# Autodesk Inventor assembly: load_cell_assembly
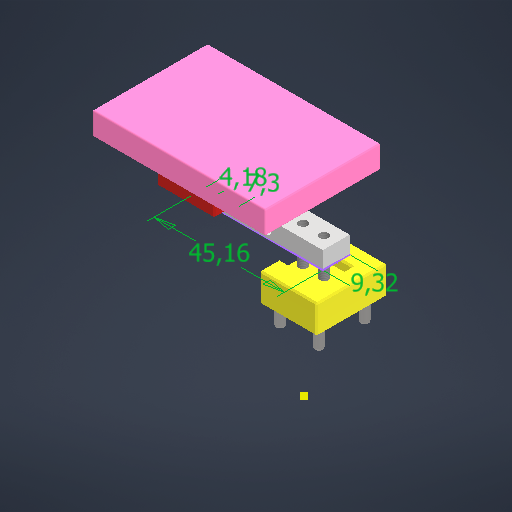
[picture p0: Inventor's stored thumbnail of the model, 512x512]
Saved by Autodesk Inventor 2026 (Build 300175000, 175)
## iProperties
Created: 2025-04-21
Part Number: load_cell_assembly
Document SubType Name: Assembly
Designer: Paul Juschitz
Author: Paul Juschitz
## Documents named in this file (8)
- C:\Users\Paul Juschitz\Documents\private\m5_GBW_mod\M5_GBW_mod\CAD\load_cell_assembly.iam
- C:\Users\Paul Juschitz\Documents\private\m5_GBW_mod\M5_GBW_mod\CAD\load_cell.ipt
- C:\Users\Paul Juschitz\Documents\private\m5_GBW_mod\M5_GBW_mod\CAD\load_cell_connector_bottom.ipt
- C:\Users\Paul Juschitz\Documents\private\m5_GBW_mod\M5_GBW_mod\CAD\load_cell_connector_top.ipt
- C:\Users\Paul Juschitz\Documents\Inventor\Content Center Files\R2026\en-US\BS EN ISO 2338\ISO 2338 - 3 h8 x 8 - B(3).ipt
- C:\Users\Paul Juschitz\Documents\Inventor\Content Center Files\R2026\en-US\AS 1237 (2.1)\AS 1237 - 3.ipt
- C:\Users\Paul Juschitz\Documents\Inventor\Content Center Files\R2026\en-US\DIN 7985 (Z)\DIN 7985 (Z) - M3x10-Z.ipt
- C:\Users\Paul Juschitz\Documents\private\m5_GBW_mod\M5_GBW_mod\CAD\plate.ipt
## Components (20 placed, 7 different names)
1. load_cell:1 — Mate:1, Mate:2, Angle:1, Mate:3, Mate:4, Cylindrical:16, Cylindrical:17, Angle:6, Angle:7, Cylindrical:18, Cylindrical:19
2. load_cell_connector_bottom:2 — Angle:1, Mate:3, Mate:4, Cylindrical:5, Cylindrical:6, Cylindrical:7, Cylindrical:8, Cylindrical:13, Cylindrical:14, Mate:9, Mate:10
3. load_cell_connector_top:1 — Mate:1, Mate:2, Cylindrical:1, Cylindrical:2, Cylindrical:3, Cylindrical:4, Angle:2, Cylindrical:9, Cylindrical:11, Mate:11, Mate:12, Mate:13, Mate:14, Mate:15, Mate:16
4. BS EN ISO 2338 3 h8 x 8 - B:1 — Cylindrical:2, Mate:16, Cylindrical:20
5. BS EN ISO 2338 3 h8 x 8 - B:2 — Cylindrical:1, Mate:15
6. BS EN ISO 2338 3 h8 x 8 - B:3 — Cylindrical:4, Mate:14, Cylindrical:21
7. BS EN ISO 2338 3 h8 x 8 - B:4 — Cylindrical:6
8. BS EN ISO 2338 3 h8 x 8 - B:5 — Cylindrical:5
9. BS EN ISO 2338 3 h8 x 8 - B:6 — Cylindrical:7
10. BS EN ISO 2338 3 h8 x 8 - B:7 — Cylindrical:8
11. BS EN ISO 2338 3 h8 x 8 - B:8 — Cylindrical:3, Mate:13
12. AS 1237 (2.1) 3:1 — Angle:2, Angle:3, Cylindrical:9, Mate:6, Mate:12
13. AS 1237 (2.1) 3:2 — Angle:3, Angle:4, Cylindrical:11, Mate:5, Mate:11
14. AS 1237 (2.1) 3:3 — Angle:4, Angle:5, Cylindrical:13, Mate:7, Mate:9
15. AS 1237 (2.1) 3:4 — Angle:5, Cylindrical:14, Mate:8, Mate:10
16. DIN 7985 (Z) M3x10-Z:1 — Cylindrical:16, Mate:7
17. DIN 7985 (Z) M3x10-Z:2 — Cylindrical:17, Mate:8
18. DIN 7985 (Z) M3x10-Z:3 — Angle:7, Cylindrical:19, Mate:6
19. DIN 7985 (Z) M3x10-Z:4 — Angle:6, Cylindrical:18, Mate:5
20. plate:1 — Cylindrical:20, Cylindrical:21
## Relationships (41: CylindricalJoint 18, Mate 16, Angle 7)
- Mate:1: load_cell:1 ↔ load_cell_connector_top:1
- Mate:2: load_cell:1 ↔ load_cell_connector_top:1
- Angle:1 (180 deg): load_cell:1 ↔ load_cell_connector_bottom:2
- Mate:3: load_cell:1 ↔ load_cell_connector_bottom:2
- Mate:4: load_cell:1 ↔ load_cell_connector_bottom:2
- Cylindrical:1: load_cell_connector_top:1 ↔ BS EN ISO 2338 3 h8 x 8 - B:2
- Cylindrical:2: load_cell_connector_top:1 ↔ BS EN ISO 2338 3 h8 x 8 - B:1
- Cylindrical:3: load_cell_connector_top:1 ↔ BS EN ISO 2338 3 h8 x 8 - B:8
- Cylindrical:4: load_cell_connector_top:1 ↔ BS EN ISO 2338 3 h8 x 8 - B:3
- Cylindrical:5: load_cell_connector_bottom:2 ↔ BS EN ISO 2338 3 h8 x 8 - B:5
- Cylindrical:6: load_cell_connector_bottom:2 ↔ BS EN ISO 2338 3 h8 x 8 - B:4
- Cylindrical:7: load_cell_connector_bottom:2 ↔ BS EN ISO 2338 3 h8 x 8 - B:6
- Cylindrical:8: load_cell_connector_bottom:2 ↔ BS EN ISO 2338 3 h8 x 8 - B:7
- Angle:2 (0 deg): load_cell_connector_top:1 ↔ AS 1237 (2.1) 3:1
- Angle:3 (0 deg): AS 1237 (2.1) 3:1 ↔ AS 1237 (2.1) 3:2
- Angle:4 (0 deg): AS 1237 (2.1) 3:2 ↔ AS 1237 (2.1) 3:3
- Angle:5 (0 deg): AS 1237 (2.1) 3:3 ↔ AS 1237 (2.1) 3:4
- Cylindrical:9: load_cell_connector_top:1 ↔ AS 1237 (2.1) 3:1
- Cylindrical:11: load_cell_connector_top:1 ↔ AS 1237 (2.1) 3:2
- Cylindrical:13: load_cell_connector_bottom:2 ↔ AS 1237 (2.1) 3:3
- Cylindrical:14: load_cell_connector_bottom:2 ↔ AS 1237 (2.1) 3:4
- Cylindrical:16: load_cell:1 ↔ DIN 7985 (Z) M3x10-Z:1
- Cylindrical:17: load_cell:1 ↔ DIN 7985 (Z) M3x10-Z:2
- Angle:6 (0 deg): load_cell:1 ↔ DIN 7985 (Z) M3x10-Z:4
- Angle:7 (0 deg): load_cell:1 ↔ DIN 7985 (Z) M3x10-Z:3
- Cylindrical:18: load_cell:1 ↔ DIN 7985 (Z) M3x10-Z:4
- Cylindrical:19: load_cell:1 ↔ DIN 7985 (Z) M3x10-Z:3
- Mate:5: AS 1237 (2.1) 3:2 ↔ DIN 7985 (Z) M3x10-Z:4
- Mate:6: AS 1237 (2.1) 3:1 ↔ DIN 7985 (Z) M3x10-Z:3
- Mate:7: AS 1237 (2.1) 3:3 ↔ DIN 7985 (Z) M3x10-Z:1
- Mate:8: AS 1237 (2.1) 3:4 ↔ DIN 7985 (Z) M3x10-Z:2
- Mate:9: load_cell_connector_bottom:2 ↔ AS 1237 (2.1) 3:3
- Mate:10: load_cell_connector_bottom:2 ↔ AS 1237 (2.1) 3:4
- Mate:11: load_cell_connector_top:1 ↔ AS 1237 (2.1) 3:2
- Mate:12: load_cell_connector_top:1 ↔ AS 1237 (2.1) 3:1
- Mate:13: load_cell_connector_top:1 ↔ BS EN ISO 2338 3 h8 x 8 - B:8
- Mate:14: load_cell_connector_top:1 ↔ BS EN ISO 2338 3 h8 x 8 - B:3
- Mate:15: load_cell_connector_top:1 ↔ BS EN ISO 2338 3 h8 x 8 - B:2
- Mate:16: load_cell_connector_top:1 ↔ BS EN ISO 2338 3 h8 x 8 - B:1
- Cylindrical:20: BS EN ISO 2338 3 h8 x 8 - B:1 ↔ plate:1
- Cylindrical:21: BS EN ISO 2338 3 h8 x 8 - B:3 ↔ plate:1
